# Autodesk Inventor assembly: Fr.wing1
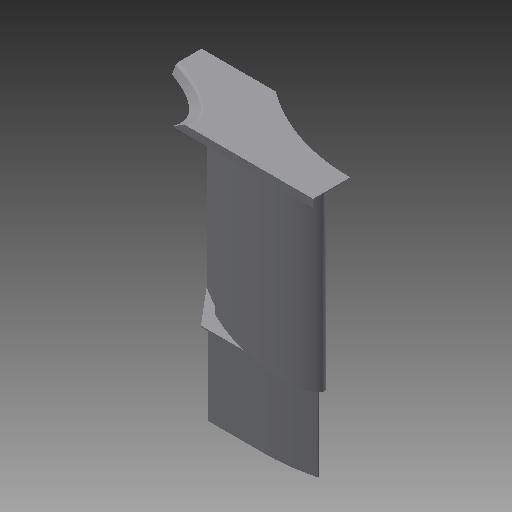
[picture p0: Inventor's stored thumbnail of the model, 512x512]
Saved by Autodesk Inventor 2018.2 (Build 222227000, 227)
## iProperties
Created: 2018-02-26
Part Number: Fr.wing1
Material: 一般
Document SubType Name: Assembly
Designer: ku_sk
Author: ku_sk
## Documents named in this file (7)
- C:\Users\ku_sk\Documents\Inventor\AeroCAD2018\設計\Fr.wing\Fr.wing1.iam
- C:\Users\ku_sk\Documents\Inventor\AeroCAD2018\設計\Fr.wing\parts\endplate1.ipt
- C:\Users\ku_sk\Documents\Inventor\AeroCAD2018\設計\Fr.wing\parts\mainflap1.ipt
- C:\Users\ku_sk\Documents\Inventor\AeroCAD2018\設計\Fr.wing\parts\subflap1.ipt
- C:\Users\ku_sk\Documents\Inventor\AeroCAD2018\設計\Fr.wing\parts\subflap21.ipt
- C:\Users\ku_sk\Documents\Inventor\AeroCAD2018\設計\Fr.wing\parts\bracket1.ipt
- C:\Users\ku_sk\Documents\Inventor\AeroCAD2018\設計\Fr.wing\parts\mainflapcenter1.ipt
## Components (6 placed, 6 different names)
1. endplate1:1 — メイト:1, メイト:2, メイト:4, メイト:5
2. mainflap1:1 — メイト:2, 角度:1, メイト:6
3. subflap1:1 — メイト:4, 角度:2
4. subflap21:1 — 角度:2, 角度:1, メイト:5
5. bracket1:1 — メイト:6, メイト:7
6. mainflapcenter1:1 — メイト:7
## Relationships (8: Mate 5, Angle 2, Flush 1)
- メイト:1 [Flush]: endplate1:1
- メイト:2 [Mate]: endplate1:1 ↔ mainflap1:1
- メイト:4 [Mate]: endplate1:1 ↔ subflap1:1
- 角度:2 [Angle] (-15 deg): subflap1:1 ↔ subflap21:1
- 角度:1 [Angle] (-15 deg): mainflap1:1 ↔ subflap21:1
- メイト:5 [Mate]: endplate1:1 ↔ subflap21:1
- メイト:6 [Mate]: mainflap1:1 ↔ bracket1:1
- メイト:7 [Mate]: bracket1:1 ↔ mainflapcenter1:1
